# Autodesk Inventor assembly: 2sr_ass_tmp
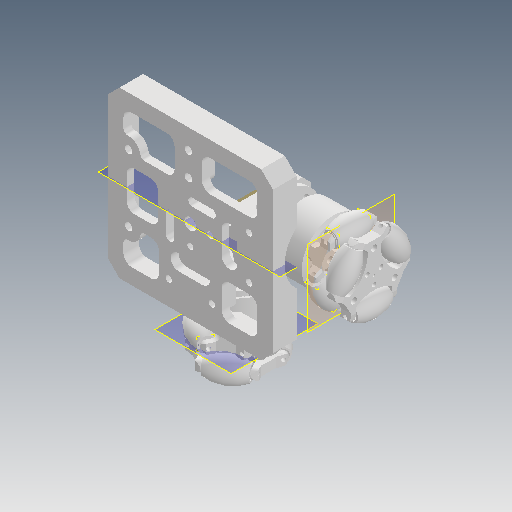
[picture p0: Inventor's stored thumbnail of the model, 512x512]
Saved by Autodesk Inventor 2020 (Build 240168000, 168)
## iProperties
Created: 2022-07-27
Part Number: 2sr_ass_tmp
Document SubType Name: Assembly
Designer: Shuang Peng
Author: Shuang Peng
## Documents named in this file (3)
- D:\projects-3\soft module robot\hardware\diff module 3\2sr_ass_tmp.iam
- D:\projects-3\soft module robot\hardware\diff module 3\base_shell_2.ipt
- D:\projects-3\soft module robot\hardware\diff module 3\base_ass_2.iam
## Components (3 placed, 2 different names)
1. base_shell_2:1 — Mate:3, Mate:4, Flush:1, Flush:2, Flush:3, Flush:4
2. base_ass_2:1 [sub-assembly] — Mate:3, Flush:2, Flush:4
3. base_ass_2:2 [sub-assembly] — Mate:4, Flush:1, Flush:3
## Relationships (6: Flush 4, Mate 2)
- Mate:3: base_shell_2:1 ↔ base_ass_2:1
- Mate:4: base_shell_2:1 ↔ base_ass_2:2
- Flush:1 (13.5 mm): base_shell_2:1 ↔ base_ass_2:2
- Flush:2 (13.5 mm): base_shell_2:1 ↔ base_ass_2:1
- Flush:3 (24.5 mm): base_shell_2:1 ↔ base_ass_2:2
- Flush:4 (24.5 mm): base_shell_2:1 ↔ base_ass_2:1
